# Autodesk Inventor assembly: Assembly_1_servo_MIR
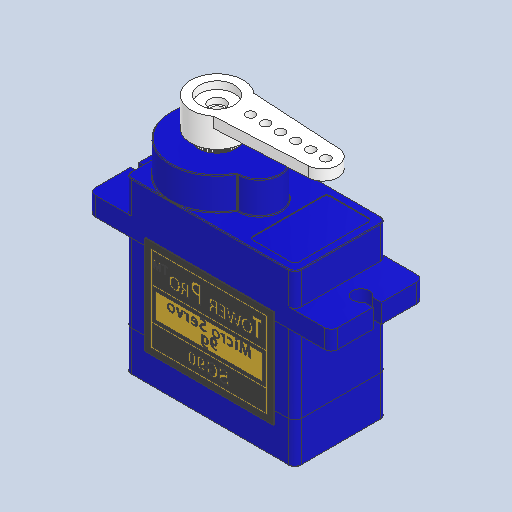
[picture p0: Inventor's stored thumbnail of the model, 512x512]
Saved by Autodesk Inventor 2023 (Build 270158000, 158)
## iProperties
Created: 2023-09-29
Part Number: Assembly_1_servo_MIR
Document SubType Name: Assembly
Designer: zskus
Author: zskus
## Documents named in this file (3)
- C:\Users\zskus\Desktop\Folders\Personal Projects\Inventor\Project_1_Scooter\Assembly\Assembly_1_servo_MIR.iam
- C:\Users\zskus\Desktop\Folders\Personal Projects\Inventor\Project_1_Scooter\Parts\SG90 - Micro Servo 9g - Tower Pro.1_MIR.ipt
- C:\Users\zskus\Desktop\Folders\Personal Projects\Inventor\Project_1_Scooter\Parts\SG90 - Micro Servo 9g - Tower Pro.2_MIR.ipt
## Components (2 placed, 2 different names)
1. SG90 - Micro Servo 9g - Tower Pro.1_MIR:1 — Mate:2, Mate:1
2. SG90 - Micro Servo 9g - Tower Pro.2_MIR:1 — Mate:2, Mate:1
## Relationships (2: Mate 2)
- Mate:2: SG90 - Micro Servo 9g - Tower Pro.1_MIR:1 ↔ SG90 - Micro Servo 9g - Tower Pro.2_MIR:1
- Mate:1: SG90 - Micro Servo 9g - Tower Pro.1_MIR:1 ↔ SG90 - Micro Servo 9g - Tower Pro.2_MIR:1
